# Autodesk Inventor assembly: ASY PNS780-Filter legs D1200
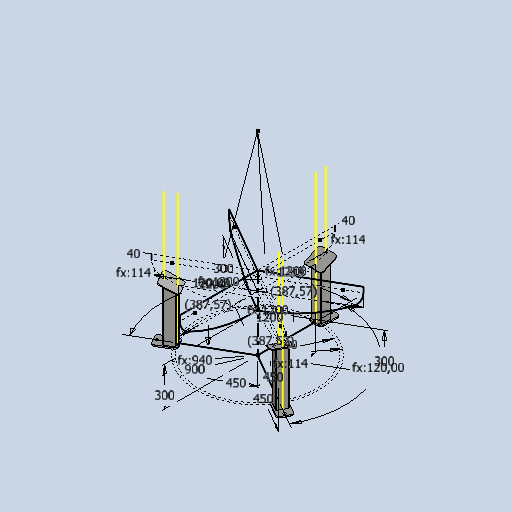
[picture p0: Inventor's stored thumbnail of the model, 512x512]
Saved by Autodesk Inventor 2025 (Build 290162010, 162A)
## iProperties
Created: 2025-02-20
Part Number: ASY PNS780-Filter legs D1200
Document SubType Name: Assembly
Designer: user
Author: user
## Documents named in this file (5)
- C:\Users\admin\YandexDisk-badmisterfox\home pc\Inventor\PNS-Panaevsk\Filter D1200\ASY PNS780-Filter legs D1200.iam
- C:\Users\admin\YandexDisk-badmisterfox\home pc\Inventor\PNS-Panaevsk\Filter D1200\PNS-781 Leg tube.ipt
- C:\Users\admin\YandexDisk-badmisterfox\home pc\Inventor\PNS-Panaevsk\Filter D1200\PNS-789 leg sketch.ipt
- C:\Users\admin\YandexDisk-badmisterfox\home pc\Inventor\PNS-Panaevsk\Filter D1200\PNS-782 leg plate for filter.ipt
- C:\Users\admin\YandexDisk-badmisterfox\home pc\Inventor\PNS-Panaevsk\Filter D1200\PNS-783 leg floor plate.ipt
## Components (10 placed, 4 different names)
1. ISO 4019 - 200x200x5 - 800.ipt:1 — Mate:2, Mate:8, Tangent:2, Rigid:2, Rigid:5
2. ISO 4019 - 200x200x5 - 800.ipt:2 — Mate:4, Mate:7, Tangent:3, Rigid:1, Rigid:4
3. ISO 4019 - 200x200x5 - 800.ipt:3 — Mate:3, Mate:6, Tangent:1, Rigid:3, Rigid:6
4. Part2ntdddasd.ipt:1 — Mate:6, Tangent:1, Mate:7, Mate:8, Tangent:2, Tangent:3
5. temp filter leg plate.ipt:1 — Rigid:1
6. temp filter leg plate.ipt:2 — Rigid:2
7. temp filter leg plate.ipt:3 — Rigid:3
8. temp filter leg plate_CPY.ipt:1 — Rigid:4
9. temp filter leg plate_CPY.ipt:2 — Rigid:5
10. temp filter leg plate_CPY.ipt:3 — Rigid:6
## Relationships (15: Mate 6, WeldJoint 6, Tangent 3)
- Mate:2: ISO 4019 - 200x200x5 - 800.ipt:1
- Mate:3: ISO 4019 - 200x200x5 - 800.ipt:3
- Mate:4: ISO 4019 - 200x200x5 - 800.ipt:2
- Mate:6: ISO 4019 - 200x200x5 - 800.ipt:3 ↔ Part2ntdddasd.ipt:1
- Tangent:1: ISO 4019 - 200x200x5 - 800.ipt:3 ↔ Part2ntdddasd.ipt:1
- Mate:7: ISO 4019 - 200x200x5 - 800.ipt:2 ↔ Part2ntdddasd.ipt:1
- Mate:8: ISO 4019 - 200x200x5 - 800.ipt:1 ↔ Part2ntdddasd.ipt:1
- Tangent:2: ISO 4019 - 200x200x5 - 800.ipt:1 ↔ Part2ntdddasd.ipt:1
- Tangent:3: ISO 4019 - 200x200x5 - 800.ipt:2 ↔ Part2ntdddasd.ipt:1
- Rigid:1 [WeldJoint]: ISO 4019 - 200x200x5 - 800.ipt:2 ↔ temp filter leg plate.ipt:1
- Rigid:2 [WeldJoint]: ISO 4019 - 200x200x5 - 800.ipt:1 ↔ temp filter leg plate.ipt:2
- Rigid:3 [WeldJoint]: ISO 4019 - 200x200x5 - 800.ipt:3 ↔ temp filter leg plate.ipt:3
- Rigid:4 [WeldJoint]: ISO 4019 - 200x200x5 - 800.ipt:2 ↔ temp filter leg plate_CPY.ipt:1
- Rigid:5 [WeldJoint]: ISO 4019 - 200x200x5 - 800.ipt:1 ↔ temp filter leg plate_CPY.ipt:2
- Rigid:6 [WeldJoint]: ISO 4019 - 200x200x5 - 800.ipt:3 ↔ temp filter leg plate_CPY.ipt:3
